# Autodesk Inventor assembly: B1F-Mirror_OnPost
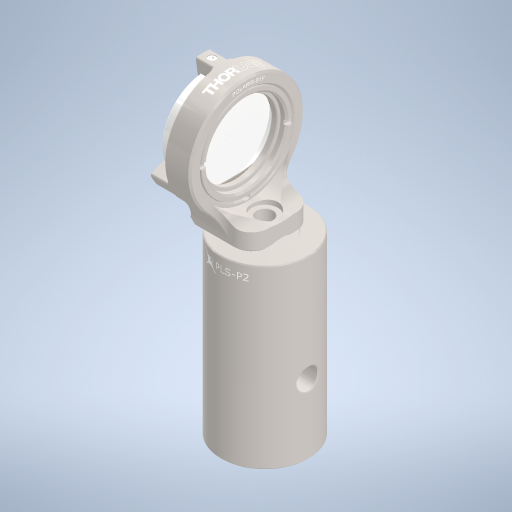
[picture p0: Inventor's stored thumbnail of the model, 512x512]
Saved by Autodesk Inventor 2024.2 (Build 282272000, 272)
## iProperties
Created: 2025-01-03
Part Number: B1F-Mirror_OnPost
Document SubType Name: Assembly
Designer: monolithic
Author: monolithic
## Documents named in this file (4)
- C:\Users\monolithic\Documents\GitHub\CAD\Monolith\John\ASLM_SampleScanning_Baseplate\Assembly\Components\SubAssemblies\B1F-Mirror_OnPost.iam
- C:\Users\monolithic\Documents\GitHub\CAD\Monolith\John\ASLM_SampleScanning_Baseplate\Assembly\Components\SubAssemblies\POLARIS-B1F.ipt
- C:\Users\monolithic\Documents\GitHub\CAD\Monolith\John\ASLM_SampleScanning_Baseplate\Assembly\Components\SubAssemblies\PF10-03-P01.ipt
- C:\Users\monolithic\Documents\GitHub\CAD\Monolith\John\ASLM_SampleScanning_Baseplate\Assembly\Components\SubAssemblies\PLS-P2.ipt
## Components (3 placed, 3 different names)
1. POLARIS-B1F:1 — Mate:1, Mate:2, Mate:3, Mate:4, Mate:5
2. PF10-03-P01:1 — Mate:1, Mate:2
3. PLS-P2:1 — Mate:3, Mate:4, Mate:5
## Relationships (5: Mate 5)
- Mate:1: POLARIS-B1F:1 ↔ PF10-03-P01:1
- Mate:2: POLARIS-B1F:1 ↔ PF10-03-P01:1
- Mate:3: POLARIS-B1F:1 ↔ PLS-P2:1
- Mate:4: POLARIS-B1F:1 ↔ PLS-P2:1
- Mate:5: POLARIS-B1F:1 ↔ PLS-P2:1
